# Autodesk Inventor assembly: 15102898-16-A-0400
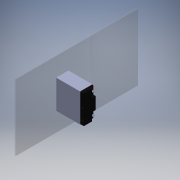
[picture p0: Inventor's stored thumbnail of the model, 180x180]
Saved by Autodesk Inventor 2017 (Build 210142000, 142)
## iProperties
Created: 2016-10-03
Part Number: 15102898-16-A-0400
Document SubType Name: Assembly
Designer: gus
Author: gus
## Documents named in this file (9)
- \\Mac\Home\Desktop\bunnybots 2016\15102898-16-Bunnybot-CAD\Bunnybot-To_be_renamed\15102898-16-A-0000\15102898-16-A-0400\15102898-16-A-0400.iam
- \\Mac\Home\Desktop\bunnybots 2016\15102898-16-Bunnybot-CAD\Bunnybot-To_be_renamed\15102898-16-A-0000\15102898-16-A-0400\15102898-16-P-0401.ipt
- \\Mac\Home\Desktop\bunnybots 2016\15102898-16-Bunnybot-CAD\Bunnybot-To_be_renamed\15102898-16-A-0000\15102898-16-A-0400\Imported Components\User Library-Battery-6.ipt
- \\Mac\Home\Desktop\bunnybots 2016\15102898-16-Bunnybot-CAD\Bunnybot-To_be_renamed\15102898-16-A-0000\15102898-16-A-0400\15102898-16-P-0402.ipt
- \\Mac\Home\Desktop\bunnybots 2016\15102898-16-Bunnybot-CAD\Bunnybot-To_be_renamed\15102898-16-A-0000\15102898-16-A-0400\15102898-16-P-0403.ipt
- \\Mac\Home\Desktop\bunnybots 2016\15102898-16-Bunnybot-CAD\Bunnybot-To_be_renamed\15102898-16-A-0000\15102898-16-A-0400\15102898-16-P-0404.ipt
- \\Mac\Home\Desktop\bunnybots 2016\15102898-16-Bunnybot-CAD\Bunnybot-To_be_renamed\15102898-16-A-0000\15102898-16-A-0400\15102898-16-P-0405.ipt
- \\Mac\Home\Desktop\bunnybots 2016\15102898-16-Bunnybot-CAD\Bunnybot-To_be_renamed\15102898-16-A-0000\15102898-16-A-0300\Imported Components\91860A029_TYPE 17-7 PH STAINLESS STEEL FLAT WASHER.ipt
- \\Mac\Home\Desktop\bunnybots 2016\15102898-16-Bunnybot-CAD\Bunnybot-To_be_renamed\15102898-16-A-0000\15102898-16-A-0300\Imported Components\92001A321_18-8 SS WING NUT.ipt
## Components (11 placed, 8 different names)
1. 15102898-16-P-0401:1 — Flush:1, Flush:2, Mate:1, Mate:4, Flush:4, Flush:5
2. User Library-Battery-6:1 — Flush:1, Flush:2, Mate:2, Flush:3, Mate:3, Mate:7
3. 15102898-16-P-0402:1 — Mate:1, Mate:2, Flush:3, Mate:3
4. 15102898-16-P-0403:1 — Mate:4, Flush:4, Flush:5, Mate:5, Flush:6, Mate:6, Flush:7
5. 15102898-16-P-0404:1 — Mate:5, Flush:6, Mate:9, Mate:13, Mate:15
6. 15102898-16-P-0404:2 — Mate:6, Flush:7, Mate:8, Mate:11, Mate:17
7. 15102898-16-P-0405:1 — Mate:7, Mate:8, Mate:9, Mate:10, Mate:12, Mate:14, Mate:16
8. 91860A029_TYPE 17-7 PH STAINLESS STEEL FLAT WASHER:1 — Mate:12, Mate:13
9. 92001A321_18-8 SS WING NUT:1 — Mate:16, Mate:17
10. 91860A029_TYPE 17-7 PH STAINLESS STEEL FLAT WASHER:2 — Mate:10, Mate:11
11. 92001A321_18-8 SS WING NUT:2 — Mate:14, Mate:15
## Relationships (24: Mate 17, Flush 7)
- Flush:1 (215.9 mm): 15102898-16-P-0401:1 ↔ User Library-Battery-6:1
- Flush:2 (114.3 mm): 15102898-16-P-0401:1 ↔ User Library-Battery-6:1
- Mate:1: 15102898-16-P-0401:1 ↔ 15102898-16-P-0402:1
- Mate:2: User Library-Battery-6:1 ↔ 15102898-16-P-0402:1
- Flush:3: User Library-Battery-6:1 ↔ 15102898-16-P-0402:1
- Mate:3: User Library-Battery-6:1 ↔ 15102898-16-P-0402:1
- Mate:4: 15102898-16-P-0401:1 ↔ 15102898-16-P-0403:1
- Flush:4: 15102898-16-P-0401:1 ↔ 15102898-16-P-0403:1
- Flush:5 (214.3125 mm): 15102898-16-P-0401:1 ↔ 15102898-16-P-0403:1
- Mate:5: 15102898-16-P-0403:1 ↔ 15102898-16-P-0404:1
- Flush:6 (-6.35 mm): 15102898-16-P-0403:1 ↔ 15102898-16-P-0404:1
- Mate:6: 15102898-16-P-0403:1 ↔ 15102898-16-P-0404:2
- Flush:7 (-6.35 mm): 15102898-16-P-0403:1 ↔ 15102898-16-P-0404:2
- Mate:7: User Library-Battery-6:1 ↔ 15102898-16-P-0405:1
- Mate:8: 15102898-16-P-0404:2 ↔ 15102898-16-P-0405:1
- Mate:9: 15102898-16-P-0404:1 ↔ 15102898-16-P-0405:1
- Mate:10: 15102898-16-P-0405:1 ↔ 91860A029_TYPE 17-7 PH STAINLESS STEEL FLAT WASHER:2
- Mate:11: 15102898-16-P-0404:2 ↔ 91860A029_TYPE 17-7 PH STAINLESS STEEL FLAT WASHER:2
- Mate:12: 15102898-16-P-0405:1 ↔ 91860A029_TYPE 17-7 PH STAINLESS STEEL FLAT WASHER:1
- Mate:13: 15102898-16-P-0404:1 ↔ 91860A029_TYPE 17-7 PH STAINLESS STEEL FLAT WASHER:1
- Mate:14: 15102898-16-P-0405:1 ↔ 92001A321_18-8 SS WING NUT:2
- Mate:15: 15102898-16-P-0404:1 ↔ 92001A321_18-8 SS WING NUT:2
- Mate:16: 15102898-16-P-0405:1 ↔ 92001A321_18-8 SS WING NUT:1
- Mate:17: 15102898-16-P-0404:2 ↔ 92001A321_18-8 SS WING NUT:1
